# Autodesk Inventor assembly: Polarizer
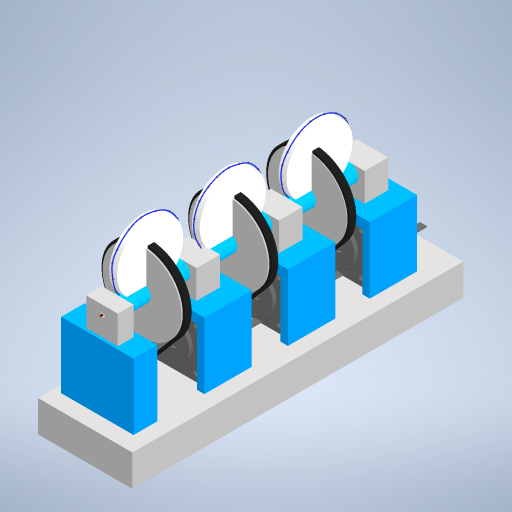
[picture p0: Inventor's stored thumbnail of the model, 512x512]
Saved by Autodesk Inventor 2024 (Build 280153000, 153)
## iProperties
Created: 2024-02-15
Part Number: Polarizer
Document SubType Name: Assembly
Designer: fabiancastano
Author: fabiancastano
## Documents named in this file (6)
- C:\GitHub\PulseLaserPrj\CaseDesign\Polarizer.iam
- C:\GitHub\PulseLaserPrj\CaseDesign\BaseFiles\Motores.ipt
- C:\GitHub\PulseLaserPrj\CaseDesign\BaseFiles\NEMA14\NEMA14.iam
- C:\GitHub\PulseLaserPrj\CaseDesign\motores\belt.ipt
- C:\GitHub\PulseLaserPrj\CaseDesign\motores\terminal.ipt
- C:\GitHub\PulseLaserPrj\CaseDesign\Polarizer\AIP\Cable and Harness\Polarizer.Harness5.iam
## Components (10 placed, 5 different names)
1. Motores:1 — Mate:1, Flush:1, Mate:2, Mate:3, Mate:4, Flush:2, Flush:3, Mate:5, Mate:6, Flush:4, Mate:7, Mate:8, Mate:9, Flush:6, Flush:7, Mate:10, Mate:11, Mate:12, Mate:13, Flush:8
2. NEMA14:1 [sub-assembly] — Mate:1, Flush:1, Mate:2, Tangent:1
3. NEMA14:2 [sub-assembly] — Mate:3, Flush:2, Mate:5, Tangent:2
4. NEMA14:3 [sub-assembly] — Mate:4, Flush:3, Mate:6, Tangent:3
5. belt:1 — Flush:5, Mate:7, Tangent:1
6. belt:2 — Mate:8, Tangent:2, Flush:6
7. belt:3 — Mate:9, Tangent:3, Flush:7
8. terminal:1 — Mate:10, Mate:11
9. terminal:2 — Mate:12, Mate:13
10. Harness5 [sub-assembly]
## Relationships (24: Mate 13, Flush 8, Tangent 3)
- Mate:1: Motores:1 ↔ NEMA14:1
- Flush:1: Motores:1 ↔ NEMA14:1
- Mate:2 (1 mm): Motores:1 ↔ NEMA14:1
- Mate:3: Motores:1 ↔ NEMA14:2
- Mate:4: Motores:1 ↔ NEMA14:3
- Flush:2: Motores:1 ↔ NEMA14:2
- Flush:3: Motores:1 ↔ NEMA14:3
- Mate:5 (1 mm): Motores:1 ↔ NEMA14:2
- Mate:6 (1 mm): Motores:1 ↔ NEMA14:3
- Flush:4 (-2.5 mm): Motores:1
- Flush:5: belt:1
- Mate:7: Motores:1 ↔ belt:1
- Tangent:1: NEMA14:1 ↔ belt:1
- Mate:8: Motores:1 ↔ belt:2
- Mate:9: Motores:1 ↔ belt:3
- Tangent:2: NEMA14:2 ↔ belt:2
- Tangent:3: NEMA14:3 ↔ belt:3
- Flush:6: Motores:1 ↔ belt:2
- Flush:7: Motores:1 ↔ belt:3
- Mate:10: Motores:1 ↔ terminal:1
- Mate:11: Motores:1 ↔ terminal:1
- Mate:12: Motores:1 ↔ terminal:2
- Mate:13: Motores:1 ↔ terminal:2
- Flush:8 (-5.25 mm): Motores:1
